# Autodesk Inventor assembly: BikeAssembly
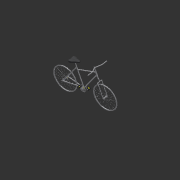
[picture p0: Inventor's stored thumbnail of the model, 180x180]
Saved by Autodesk Inventor 2019 (Build 230136000, 136)
## iProperties
Created: 2020-01-15
Part Number: BikeAssembly
Document SubType Name: Assembly
Designer: 18186
Author: 18186
## Documents named in this file (21)
- C:\Users\18186\Desktop\Important Shit\Michael Goldberg Portfolio\CAD Portfolio\IPT Files\Bike\BikeAssembly.iam
- C:\Users\18186\Desktop\Important Shit\Michael Goldberg Portfolio\CAD Portfolio\IPT Files\Bike\Bike Frame.ipt
- C:\Users\18186\Desktop\Important Shit\Michael Goldberg Portfolio\CAD Portfolio\IPT Files\Bike\Bearing.ipt
- C:\Users\18186\Desktop\Important Shit\Michael Goldberg Portfolio\CAD Portfolio\IPT Files\Bike\Fork.ipt
- C:\Users\18186\Desktop\Important Shit\Michael Goldberg Portfolio\CAD Portfolio\IPT Files\Bike\Bike Wheel.ipt
- C:\Users\18186\Desktop\Important Shit\Michael Goldberg Portfolio\CAD Portfolio\IPT Files\Bike\Bike Wheel Back.ipt
- C:\Users\18186\Desktop\Important Shit\Michael Goldberg Portfolio\CAD Portfolio\IPT Files\Bike\Bike Seat.ipt
- C:\Users\18186\Desktop\Important Shit\Michael Goldberg Portfolio\CAD Portfolio\IPT Files\Bike\Bike Seat Bolt.ipt
- C:\Users\18186\Desktop\Important Shit\Michael Goldberg Portfolio\CAD Portfolio\IPT Files\Bike\Pedal Axle.ipt
- C:\Users\18186\Desktop\Important Shit\Michael Goldberg Portfolio\CAD Portfolio\IPT Files\Bike\Pedal Shaft Extender Right.ipt
- C:\Users\18186\Desktop\Important Shit\Michael Goldberg Portfolio\CAD Portfolio\IPT Files\Bike\Pedal Shaft Extender Left.ipt
- C:\Users\18186\Desktop\Important Shit\Michael Goldberg Portfolio\CAD Portfolio\IPT Files\Bike\Pedal Crank Right.ipt
- C:\Users\18186\Desktop\Important Shit\Michael Goldberg Portfolio\CAD Portfolio\IPT Files\Bike\Pedal Crank Left.ipt
- C:\Users\18186\Desktop\Important Shit\Michael Goldberg Portfolio\CAD Portfolio\IPT Files\Bike\Pedal Assembly Right.iam
- C:\Users\18186\Desktop\Important Shit\Michael Goldberg Portfolio\CAD Portfolio\IPT Files\Bike\Pedal Bolt Outside Right.ipt
- C:\Users\18186\Desktop\Important Shit\Michael Goldberg Portfolio\CAD Portfolio\IPT Files\Bike\Pedal Assembly Left.iam
- C:\Users\18186\Desktop\Important Shit\Michael Goldberg Portfolio\CAD Portfolio\IPT Files\Bike\Pedal Bolt Outside Left.ipt
- C:\Users\18186\Desktop\Important Shit\Michael Goldberg Portfolio\CAD Portfolio\IPT Files\Bike\Pedal Bar.ipt
- C:\Users\18186\Desktop\Important Shit\Michael Goldberg Portfolio\CAD Portfolio\IPT Files\Bike\Pedal Bar Bolt.ipt
- C:\Users\18186\Desktop\Important Shit\Michael Goldberg Portfolio\CAD Portfolio\IPT Files\Bike\Pedal Bar Nut.ipt
- C:\Users\18186\Desktop\Important Shit\Michael Goldberg Portfolio\CAD Portfolio\IPT Files\Bike\chain path.ipt
## Components (27 placed, 20 different names)
1. Bike Frame:1 — Mate:2, Mate:26, Mate:27, Mate:28, Mate:30, Mate:44, Mate:45, Mate:48, Mate:52, Tangent:1, Mate:55, Mate:56, Mate:82, Tangent:4, Mate:84
2. Fork:1 — Mate:2, Mate:42, Mate:43, Mate:48
3. Bearing:15 — Mate:26, Mate:27, Mate:47
4. Bearing:16 — Mate:44, Mate:45, Mate:46
5. Bearing:17 — Mate:28, Mate:55, Mate:57, Flush:1, Mate:59
6. Bearing:18 — Mate:30, Mate:56, Mate:61
7. Bearing:23 — Mate:40, Mate:41, Mate:42, Mate:43
8. Bearing:24 — Mate:38, Mate:39
9. Bike Wheel:5 — Mate:38, Mate:39, Mate:40, Mate:41
10. Bike Wheel Back:1 — Mate:46, Mate:47
11. Bike Seat:1 — Mate:82, Tangent:4
12. Bike Seat Bolt:1 — Mate:52, Tangent:1
13. Pedal Axle:1 — Mate:57, Flush:1, Mate:58, Flush:2, Mate:60, Flush:3
14. Pedal Shaft Extender Right:1 — Mate:58, Mate:59, Flush:2, Flush:4, Mate:62, Mate:63, Flush:6, Mate:85, Mate:88
15. Pedal Shaft Extender Left:1 — Mate:60, Mate:61, Flush:3, Flush:5, Mate:64, Mate:65
16. Pedal Crank Right:1 — Flush:4, Mate:62, Mate:63, Mate:66, Mate:67, Mate:68, Tangent:2, Mate:72, Mate:73
17. Pedal Crank Left:1 — Flush:5, Mate:64, Mate:65, Mate:69, Mate:70, Mate:71, Tangent:3
18. Pedal Assembly Right:1 [sub-assembly] — Mate:66, Mate:67
19. Pedal Bolt Outside Right:1 — Mate:68, Tangent:2
20. Pedal Assembly Left:1 [sub-assembly] — Mate:69, Mate:70
21. Pedal Bolt Outside Left:1 — Mate:71, Tangent:3
22. Pedal Bar:1 — Mate:72, Mate:73, Flush:6, Mate:74, Mate:75, Mate:76, Mate:77, Mate:79, Mate:81
23. Pedal Bar Bolt:1 — Mate:74, Mate:75, Mate:78
24. Pedal Bar Bolt:2 — Mate:76, Mate:77, Mate:80
25. Pedal Bar Nut:1 — Mate:78, Mate:79
26. Pedal Bar Nut:2 — Mate:80, Mate:81
27. chain path:1 — Mate:86, Mate:87, Mate:88
## Relationships (60: Mate 50, Flush 6, Tangent 4)
- Mate:2: Bike Frame:1 ↔ Fork:1
- Mate:26: Bike Frame:1 ↔ Bearing:15
- Mate:27: Bike Frame:1 ↔ Bearing:15
- Mate:28: Bike Frame:1 ↔ Bearing:17
- Mate:30: Bike Frame:1 ↔ Bearing:18
- Mate:38: Bearing:24 ↔ Bike Wheel:5
- Mate:39: Bearing:24 ↔ Bike Wheel:5
- Mate:40: Bearing:23 ↔ Bike Wheel:5
- Mate:41: Bearing:23 ↔ Bike Wheel:5
- Mate:42: Fork:1 ↔ Bearing:23
- Mate:43: Fork:1 ↔ Bearing:23
- Mate:44: Bike Frame:1 ↔ Bearing:16
- Mate:45: Bike Frame:1 ↔ Bearing:16
- Mate:46: Bearing:16 ↔ Bike Wheel Back:1
- Mate:47: Bearing:15 ↔ Bike Wheel Back:1
- Mate:48: Bike Frame:1 ↔ Fork:1
- Mate:52: Bike Frame:1 ↔ Bike Seat Bolt:1
- Tangent:1: Bike Frame:1 ↔ Bike Seat Bolt:1
- Mate:55: Bike Frame:1 ↔ Bearing:17
- Mate:56: Bike Frame:1 ↔ Bearing:18
- Mate:57: Bearing:17 ↔ Pedal Axle:1
- Flush:1 (-12.7 mm): Bearing:17 ↔ Pedal Axle:1
- Mate:58: Pedal Axle:1 ↔ Pedal Shaft Extender Right:1
- Mate:59: Bearing:17 ↔ Pedal Shaft Extender Right:1
- Flush:2: Pedal Axle:1 ↔ Pedal Shaft Extender Right:1
- Mate:60: Pedal Axle:1 ↔ Pedal Shaft Extender Left:1
- Mate:61: Bearing:18 ↔ Pedal Shaft Extender Left:1
- Flush:3: Pedal Axle:1 ↔ Pedal Shaft Extender Left:1
- Flush:4: Pedal Shaft Extender Right:1 ↔ Pedal Crank Right:1
- Mate:62: Pedal Shaft Extender Right:1 ↔ Pedal Crank Right:1
- Mate:63: Pedal Shaft Extender Right:1 ↔ Pedal Crank Right:1
- Flush:5: Pedal Shaft Extender Left:1 ↔ Pedal Crank Left:1
- Mate:64: Pedal Shaft Extender Left:1 ↔ Pedal Crank Left:1
- Mate:65: Pedal Shaft Extender Left:1 ↔ Pedal Crank Left:1
- Mate:66: Pedal Crank Right:1 ↔ Pedal Assembly Right:1
- Mate:67: Pedal Crank Right:1 ↔ Pedal Assembly Right:1
- Mate:68: Pedal Crank Right:1 ↔ Pedal Bolt Outside Right:1
- Tangent:2: Pedal Crank Right:1 ↔ Pedal Bolt Outside Right:1
- Mate:69: Pedal Crank Left:1 ↔ Pedal Assembly Left:1
- Mate:70: Pedal Crank Left:1 ↔ Pedal Assembly Left:1
- Mate:71: Pedal Crank Left:1 ↔ Pedal Bolt Outside Left:1
- Tangent:3: Pedal Crank Left:1 ↔ Pedal Bolt Outside Left:1
- Mate:72: Pedal Crank Right:1 ↔ Pedal Bar:1
- Mate:73: Pedal Crank Right:1 ↔ Pedal Bar:1
- Flush:6 (-10.16 mm): Pedal Shaft Extender Right:1 ↔ Pedal Bar:1
- Mate:74: Pedal Bar:1 ↔ Pedal Bar Bolt:1
- Mate:75: Pedal Bar:1 ↔ Pedal Bar Bolt:1
- Mate:76: Pedal Bar:1 ↔ Pedal Bar Bolt:2
- Mate:77: Pedal Bar:1 ↔ Pedal Bar Bolt:2
- Mate:78: Pedal Bar Bolt:1 ↔ Pedal Bar Nut:1
- Mate:79: Pedal Bar:1 ↔ Pedal Bar Nut:1
- Mate:80: Pedal Bar Bolt:2 ↔ Pedal Bar Nut:2
- Mate:81: Pedal Bar:1 ↔ Pedal Bar Nut:2
- Mate:82: Bike Frame:1 ↔ Bike Seat:1
- Tangent:4: Bike Frame:1 ↔ Bike Seat:1
- Mate:84: Bike Frame:1
- Mate:85: Pedal Shaft Extender Right:1
- Mate:86: chain path:1
- Mate:87: chain path:1
- Mate:88: Pedal Shaft Extender Right:1 ↔ chain path:1
